# Autodesk Inventor assembly: FinalAssembly
(part 3 of 3)
- Mate:1106: NarrowHexNutThread_5_40:209 ↔ aftServoSectionThreadedRodThread_5_40:2
- Mate:1107: NarrowHexNutThread_5_40:210 ↔ aftServoSectionThreadedRodThread_5_40:2
- Angle:78 (0 deg): NarrowHexNutThread_5_40:209 ↔ NarrowHexNutThread_5_40:210
- Angle:79 (0 deg): ServoWithShaftAssembly:1 ↔ NarrowHexNutThread_5_40:210
- Mate:1108: NarrowHexNutThread_5_40:209 ↔ HallEffectSpoolSensorMount2:1
- Flush:502 (1.905 mm): ServoWithShaftAssembly:1 ↔ HallEffectSpoolSensorMount2:1
- Mate:1110: NarrowHexNutThread_5_40:210 ↔ HallEffectSpoolSensorMount2:1
- Angle:80 (-20 deg): ServoWithShaftAssembly:1 ↔ HallEffectSpoolSensorMount2:1
- Mate:1111: HallEffectSpoolSensorMount2:1 ↔ HallEffectSensor:1
- Flush:503: HallEffectSpoolSensorMount2:1 ↔ HallEffectSensor:1
- Mate:1112: HallEffectSpoolSensorMount2:1 ↔ HallEffectSensor:1
- Mate:1113: HallEffectSpoolSensorMount2:1 ↔ aftServoSectionThreadedRodThread_5_40:2
- Flush:504: largeIdlerPinion:4 ↔ smallIdlerPinion:7
- Mate:1114 (6.096 mm): frontServoAttachmentPlate:1 ↔ largeIdlerPinion:4
- Flush:505 (2.54 mm): CarriageConnectorShaft:1 ↔ smallIdlerPinion:8
- Mate:1115: largeIdlerPinion:4 ↔ SpoolCarrageMagnetMountREV2:1
- Mate:1116: largeIdlerPinion:4 ↔ SpoolCarrageMagnetMountREV2:1
- Mate:1117: SpoolCarrageMagnetMountREV2:1 ↔ EncoderMagnet:3
- Mate:1118: SpoolCarrageMagnetMountREV2:1 ↔ EncoderMagnet:3
- Mate:1120: HallEffectSpoolSensorMount3Brace:1 ↔ aftServoSectionThreadedRodThread_5_40:6
- Mate:1121: HallEffectSpoolSensorMount3Brace:1 ↔ aftServoSectionThreadedRodThread_5_40:5
- Mate:1122: HallEffectSpoolSensorMount3:1 ↔ HallEffectSpoolSensorMount3Brace:1
- Mate:1123: HallEffectSpoolSensorMount3:1 ↔ HallEffectSpoolSensorMount3Brace:1
- Mate:1124: NarrowHexNutThread_5_40:211 ↔ aftServoSectionThreadedRodThread_5_40:5
- Mate:1125: HallEffectSpoolSensorMount3Brace:1 ↔ NarrowHexNutThread_5_40:211
- Mate:1126: NarrowHexNutThread_5_40:212 ↔ aftServoSectionThreadedRodThread_5_40:5
- Mate:1127: HallEffectSpoolSensorMount3Brace:1 ↔ NarrowHexNutThread_5_40:212
- Angle:81 (0 deg): NarrowHexNutThread_5_40:211 ↔ NarrowHexNutThread_5_40:212
- Angle:82 (0 deg): HitecServoAssembly:1 ↔ NarrowHexNutThread_5_40:211
- Mate:1128 (12.7 mm): frontServoAttachmentPlate:1 ↔ HallEffectSpoolSensorMount3Brace:1
- Mate:1129: HallEffectSpoolSensorMount3Brace:1 ↔ Bolt_ButtonHead_Hex_Thread_M3_10mm:4
- Mate:1130: HallEffectSpoolSensorMount3:1 ↔ Bolt_ButtonHead_Hex_Thread_M3_10mm:4
- Angle:83 (0 deg): HallEffectSpoolSensorMount3:1 ↔ Bolt_ButtonHead_Hex_Thread_M3_10mm:4
- Mate:1131: Bolt_ButtonHead_Hex_Thread_M3_10mm:4 ↔ HexNutThread_M3:6
- Mate:1132: HallEffectSpoolSensorMount3Brace:1 ↔ HexNutThread_M3:6
- Angle:84 (0 deg): HitecServoAssembly:2 ↔ HexNutThread_M3:6
- Mate:1133: HallEffectSpoolSensorMount3:1 ↔ HallEffectSensor:2
- Mate:1134: HallEffectSpoolSensorMount3:1 ↔ HallEffectSensor:2
- Flush:506: HallEffectSpoolSensorMount3:1 ↔ HallEffectSensor:2
- Angle:85 (0 deg): pistonSealingWallRear:1
- Angle:86 (0 deg): pistonSealingWallFront:1
- Mate:1135: ThrustBearingMount:1 ↔ HallEffectSpoolSensorMount3:2
- Mate:1136: ThrustBearingMount:1 ↔ HallEffectSpoolSensorMount3:2
- Mate:1137: HallEffectSpoolSensorMount3:2 ↔ ScrewPlastic_4_20_.5inch:38
- Mate:1138: HallEffectSpoolSensorMount3:2 ↔ ScrewPlastic_4_20_.5inch:38
- Angle:87 (0 deg): limitSwitchHolder2:1 ↔ HallEffectSpoolSensorMount3:2
- Mate:1139: NarrowHexNutThread_5_40:213 ↔ midshipsThreadedRodThread_5_40:6
- Mate:1140: ArduinoNanoHolder:1 ↔ NarrowHexNutThread_5_40:213
- Angle:88 (0 deg): ArduinoNanoHolder:1 ↔ NarrowHexNutThread_5_40:213
- Mate:1141: NarrowHexNutThread_5_40:214 ↔ midshipsThreadedRodThread_5_40:1
- Mate:1142: ArduinoNanoHolder:1 ↔ NarrowHexNutThread_5_40:214
- Angle:89 (0 deg): ArduinoNanoHolder:1 ↔ NarrowHexNutThread_5_40:214
- Mate:1143: RelayHolderREV2:1 ↔ midshipsThreadedRodThread_5_40:1
- Mate:1144: RelayHolderREV2:1 ↔ midshipsThreadedRodThread_5_40:6
- Mate:1145: RelayHolderREV2:1 ↔ RelayModule:1
- Mate:1146: RelayHolderREV2:1 ↔ RelayModule:1
- Angle:90 (0 deg): RelayHolderREV2:1 ↔ RelayModule:1
- Mate:1147: FixedCylinderWireStorage:1 ↔ SlipRingAssy:1
- Mate:1148 (9.525 mm): SpoolSectionSealingWallFront:1 ↔ SlipRingAssy:1
## Named parameters: d30_d28 = 0 mm, d31_d29 = 0 mm
